# Autodesk Inventor assembly: forest_v4_assem01
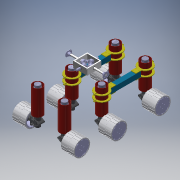
[picture p0: Inventor's stored thumbnail of the model, 180x180]
Saved by Autodesk Inventor 2018 (Build 220112000, 112)
## iProperties
Created: 2017-10-24
Part Number: forest_v4_assem01
Material: 一般
Document SubType Name: Assembly
Designer: 翔
Author: 翔
## Documents named in this file (5)
- E:\forest_robot_cad\Forest_v4\forest_v4_assem01.iam
- E:\forest_robot_cad\Forest_v4\Diffbox\Diffbox_v2.iam
- E:\forest_robot_cad\Forest_v4\holder_rocker_shaft.ipt
- E:\forest_robot_cad\Forest_v4\wheel\motor_set01.iam
- E:\forest_robot_cad\Forest_v4\bogie.iam
## Components (7 placed, 4 different names)
1. Diffbox_v2:1 [sub-assembly] — メイト:1, フラッシュ:1, メイト:2, フラッシュ:2
2. holder_rocker_shaft:1 — メイト:1, フラッシュ:1
3. holder_rocker_shaft:2 — メイト:2, フラッシュ:2
4. motor_set01:1 [sub-assembly]
5. motor_set01:4 [sub-assembly]
6. bogie:1 [sub-assembly]
7. bogie:2 [sub-assembly]
## Relationships (4: Mate 2, Flush 2)
- メイト:1 [Mate]: Diffbox_v2:1 ↔ holder_rocker_shaft:1
- フラッシュ:1 [Flush]: Diffbox_v2:1 ↔ holder_rocker_shaft:1
- メイト:2 [Mate]: Diffbox_v2:1 ↔ holder_rocker_shaft:2
- フラッシュ:2 [Flush]: Diffbox_v2:1 ↔ holder_rocker_shaft:2
